# Autodesk Inventor assembly: KON_Nietmaschine_Hebel
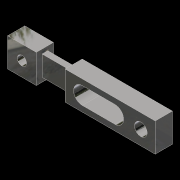
[picture p0: Inventor's stored thumbnail of the model, 180x180]
Saved by Autodesk Inventor 2019 (Build 230136000, 136)
## iProperties
Created: 2021-12-14
Part Number: KON_Nietmaschine_Hebel
Material: Generisch
Document SubType Name: Weldment
Designer: Jonas Nebl
Weld Material: Welded Aluminum-6061
Mass: 1868.76 g
Surface Area: 481.527 cm^2
Volume: 238.058 cm^3
Density: 7.85 g/cm^3
Author: Jonas Nebl
## Documents named in this file (4)
- C:\Users\jonas\Documents\Inventor\Nietmaschine\KON_Nietmaschine_Hebel.iam
- C:\Users\jonas\Documents\Inventor\Nietmaschine\EN 10058 - 50 x 30 - 157.ipt
- C:\Users\jonas\Documents\Inventor\Nietmaschine\EN 10058 - 35 x 10 - 493.ipt
- C:\Users\jonas\Documents\Inventor\Nietmaschine\EN 10058 - 50 x 30 - 50.ipt
## Components (3 placed, 3 different names)
1. EN 10058 - 50 x 30 - 157:2 — Passend:1, Fluchtend:1, Fluchtend:2, Fluchtend:3, Fluchtend:4
2. EN 10058 - 35 x 10 - 493:2 — Passend:1, Fluchtend:1, Fluchtend:2, Passend:2
3. EN 10058 - 50 x 30 - 50:1 — Passend:2, Fluchtend:3, Fluchtend:4
## Relationships (6: Flush 4, Mate 2)
- Passend:1 [Mate]: EN 10058 - 50 x 30 - 157:2 ↔ EN 10058 - 35 x 10 - 493:2
- Fluchtend:1 [Flush] (7.5 mm): EN 10058 - 50 x 30 - 157:2 ↔ EN 10058 - 35 x 10 - 493:2
- Fluchtend:2 [Flush] (10 mm): EN 10058 - 50 x 30 - 157:2 ↔ EN 10058 - 35 x 10 - 493:2
- Passend:2 [Mate]: EN 10058 - 35 x 10 - 493:2 ↔ EN 10058 - 50 x 30 - 50:1
- Fluchtend:3 [Flush]: EN 10058 - 50 x 30 - 157:2 ↔ EN 10058 - 50 x 30 - 50:1
- Fluchtend:4 [Flush]: EN 10058 - 50 x 30 - 157:2 ↔ EN 10058 - 50 x 30 - 50:1
